# Autodesk Inventor assembly: The_Assembly
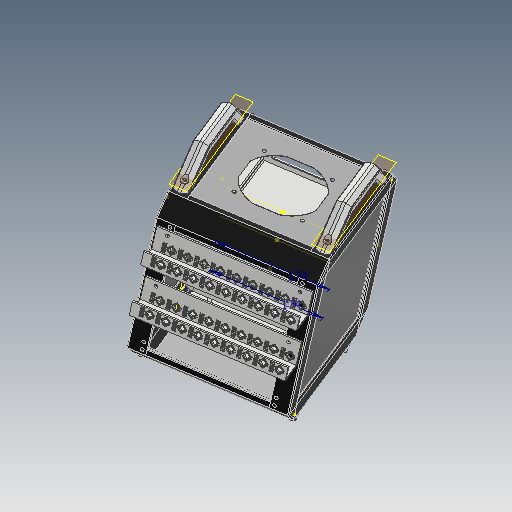
[picture p0: Inventor's stored thumbnail of the model, 512x512]
Saved by Autodesk Inventor 2027 (Build 310192060, 192F)
## iProperties
Created: 2026-07-27
Part Number: The_Assembly
Document SubType Name: Assembly
Designer: prest
Author: prest
## Documents named in this file (17)
- C:\Users\prest\OneDrive\Documents\Projects\Home_Lab_Rack\The_Assembly.iam
- C:\Users\prest\OneDrive\Documents\Projects\Home_Lab_Rack\angles_struts.ipt
- C:\Users\prest\OneDrive\Documents\Projects\Home_Lab_Rack\bottom_edge.ipt
- C:\Users\prest\OneDrive\Documents\Projects\Home_Lab_Rack\horizontal_Edge.ipt
- C:\Users\prest\OneDrive\Documents\Inventor\Content Center Files\R2027\en-US\ANSI B18.3.4M(1)\ANSI B18.3.4M - M6 x 1 x 8(2).ipt
- C:\Users\prest\OneDrive\Documents\Projects\Home_Lab_Rack\mini_PC_mount.ipt
- C:\Users\prest\OneDrive\Documents\Projects\Home_Lab_Rack\router_mount.ipt
- C:\Users\prest\OneDrive\Documents\Projects\Home_Lab_Rack\side_panel_actual.ipt
- C:\Users\prest\OneDrive\Documents\Projects\Home_Lab_Rack\bottom_panel.ipt
- C:\Users\prest\OneDrive\Documents\Projects\Home_Lab_Rack\front_panel_mount_end.ipt
- C:\Users\prest\OneDrive\Documents\Projects\Home_Lab_Rack\top panel.ipt
- C:\Users\prest\OneDrive\Documents\Projects\Home_Lab_Rack\feet.ipt
- C:\Users\prest\OneDrive\Documents\Projects\Home_Lab_Rack\top_edge.ipt
- C:\Users\prest\OneDrive\Documents\Inventor\Content Center Files\R2027\en-US\ASME ANSI B18.3.5M(2)\ASME_ANSI B18.3.5M - M6x20(2).ipt
- C:\Users\prest\OneDrive\Documents\Projects\Home_Lab_Rack\Handle.ipt
- C:\Users\prest\OneDrive\Documents\Inventor\Content Center Files\R2027\en-US\ANSI B18.3.4M(1)\ANSI B18.3.4M - M6 x 1 x 16(2).ipt
- C:\Users\prest\OneDrive\Documents\Projects\Home_Lab_Rack\cable_basket.ipt
## Components (54 placed, 16 different names)
1. Handle:3 — Rigid:21, Rigid:23, Rigid:26
2. Handle:4 — Rigid:22, Rigid:24, Rigid:25
3. Broached Hexagon Socket Button Head Cap Screw - Metric M6 x 1 x 16:1 — Rigid:23
4. Broached Hexagon Socket Button Head Cap Screw - Metric M6 x 1 x 16:2 — Rigid:24
5. Broached Hexagon Socket Button Head Cap Screw - Metric M6 x 1 x 16:3 — Rigid:25
6. Broached Hexagon Socket Button Head Cap Screw - Metric M6 x 1 x 16:4 — Rigid:26
7. cable_basket:1 — Rotational:22, Mate:30
8. cable_basket:2 — Rotational:23, Mate:31
9. Broached Hexagon Socket Flat Countersunk Head Cap Screws - Metric M6x20:1 — Flush:1, Mate:29
10. Broached Hexagon Socket Flat Countersunk Head Cap Screws - Metric M6x20:2 — Mate:27, Mate:28
11. Broached Hexagon Socket Flat Countersunk Head Cap Screws - Metric M6x20:3 — Flush:3, Mate:25
12. Broached Hexagon Socket Flat Countersunk Head Cap Screws - Metric M6x20:4 — Flush:2, Mate:26
13. Broached Hexagon Socket Button Head Cap Screw - Metric M6 x 1 x 8:1 — Rotational:1
14. Broached Hexagon Socket Button Head Cap Screw - Metric M6 x 1 x 8:2 — Rotational:2
15. Broached Hexagon Socket Button Head Cap Screw - Metric M6 x 1 x 8:3 — Rotational:3
16. Broached Hexagon Socket Button Head Cap Screw - Metric M6 x 1 x 8:4 — Rotational:5
17. Broached Hexagon Socket Button Head Cap Screw - Metric M6 x 1 x 8:5 — Rotational:6
18. Broached Hexagon Socket Button Head Cap Screw - Metric M6 x 1 x 8:6 — Rotational:4
19. Broached Hexagon Socket Button Head Cap Screw - Metric M6 x 1 x 8:7 — Rotational:7
20. Broached Hexagon Socket Button Head Cap Screw - Metric M6 x 1 x 8:8 — Rotational:8
21. Broached Hexagon Socket Button Head Cap Screw - Metric M6 x 1 x 8:13 — Rotational:14
22. Broached Hexagon Socket Button Head Cap Screw - Metric M6 x 1 x 8:14 — Rotational:15
23. Broached Hexagon Socket Button Head Cap Screw - Metric M6 x 1 x 8:15 — Rotational:16
24. Broached Hexagon Socket Button Head Cap Screw - Metric M6 x 1 x 8:17 — Rotational:17
25. Broached Hexagon Socket Button Head Cap Screw - Metric M6 x 1 x 8:18 — Rotational:19
26. Broached Hexagon Socket Button Head Cap Screw - Metric M6 x 1 x 8:19 — Rotational:18
27. Broached Hexagon Socket Button Head Cap Screw - Metric M6 x 1 x 8:20 — Rotational:20
28. Broached Hexagon Socket Button Head Cap Screw - Metric M6 x 1 x 8:21 — Rotational:21
29. angles_struts:1 — Rigid:9, Rotational:15, Rotational:16, Rotational:18, Rotational:19, Mate:13, Rigid:16, Mate:19, Mate:20, Mate:22, Mate:24
30. angles_struts:2 — Rigid:10, Rotational:14, Rotational:17, Rotational:20, Rotational:21, Mate:21, Mate:23
31. angles_struts:3 — Rigid:3, Rigid:4, Rigid:5, Rotational:1, Rotational:2, Rotational:5, Rotational:6
32. angles_struts:4 — Rigid:1, Rigid:2, Rigid:6, Rigid:7, Rotational:3, Rotational:4, Rotational:7, Rotational:8, Mate:16
33. horizontal_Edge:1 — Rigid:7, Rigid:9, Mate:1, Mate:2, Mate:4, Mate:5, Mate:8, Mate:11, Mate:14, Mate:17
34. horizontal_Edge:2 — Rigid:4, Rotational:22, Rotational:23
35. horizontal_Edge:3 — Rigid:5, Rigid:10, Mate:30, Mate:31
36. horizontal_Edge:4 — Rigid:6, Mate:3, Mate:6, Mate:7, Mate:9, Mate:10, Mate:12, Mate:15, Mate:18
37. bottom_edge:2 — Rigid:1, Rigid:3, Rigid:17, Rigid:18
38. top panel:1 — Rigid:16
39. bottom_edge:3 — Rigid:2, Rigid:15, Rigid:19, Rigid:20
40. top_edge:1 — Mate:22, Mate:23, Mate:24, Rigid:22, Rigid:28
41. top_edge:2 — Mate:19, Mate:20, Mate:21, Rigid:21, Rigid:27
42. feet:1 — Rigid:18, Mate:27, Mate:28
43. feet:2 — Rigid:17, Flush:1, Mate:29
44. feet:3 — Rigid:20, Flush:2, Mate:26
45. feet:4 — Rigid:19, Flush:3, Mate:25
46. mini_PC_mount:1 — Mate:1, Mate:2, Mate:3
47. mini_PC_mount:2 — Mate:4, Mate:5, Mate:6
48. router_mount:1 — Mate:10, Mate:11, Mate:12
49. router_mount:2 — Mate:7, Mate:8, Mate:9
50. side_panel_actual:2 — Rigid:28
51. bottom_panel:1 — Rigid:15
52. side_panel_actual:1 — Rigid:27
53. front_panel_mount_end:2 — Mate:16, Mate:17, Mate:18
54. front_panel_mount_end:1 — Mate:13, Mate:14, Mate:15
## Relationships (75: Mate 31, WeldJoint 23, RevoluteJoint 18, Flush 3)
- Rigid:1 [WeldJoint]: angles_struts:4 ↔ bottom_edge:2
- Rigid:2 [WeldJoint]: angles_struts:4 ↔ bottom_edge:3
- Rigid:3 [WeldJoint]: angles_struts:3 ↔ bottom_edge:2
- Rigid:4 [WeldJoint]: angles_struts:3 ↔ horizontal_Edge:2
- Rigid:5 [WeldJoint]: angles_struts:3 ↔ horizontal_Edge:3
- Rigid:6 [WeldJoint]: angles_struts:4 ↔ horizontal_Edge:4
- Rigid:7 [WeldJoint]: angles_struts:4 ↔ horizontal_Edge:1
- Rotational:1 [RevoluteJoint]: Broached Hexagon Socket Button Head Cap Screw - Metric M6 x 1 x 8:1 ↔ angles_struts:3
- Rotational:2 [RevoluteJoint]: Broached Hexagon Socket Button Head Cap Screw - Metric M6 x 1 x 8:2 ↔ angles_struts:3
- Rotational:3 [RevoluteJoint]: Broached Hexagon Socket Button Head Cap Screw - Metric M6 x 1 x 8:3 ↔ angles_struts:4
- Rotational:4 [RevoluteJoint]: Broached Hexagon Socket Button Head Cap Screw - Metric M6 x 1 x 8:6 ↔ angles_struts:4
- Rotational:5 [RevoluteJoint]: Broached Hexagon Socket Button Head Cap Screw - Metric M6 x 1 x 8:4 ↔ angles_struts:3
- Rotational:6 [RevoluteJoint]: Broached Hexagon Socket Button Head Cap Screw - Metric M6 x 1 x 8:5 ↔ angles_struts:3
- Rotational:7 [RevoluteJoint]: Broached Hexagon Socket Button Head Cap Screw - Metric M6 x 1 x 8:7 ↔ angles_struts:4
- Rotational:8 [RevoluteJoint]: Broached Hexagon Socket Button Head Cap Screw - Metric M6 x 1 x 8:8 ↔ angles_struts:4
- Rigid:9 [WeldJoint]: angles_struts:1 ↔ horizontal_Edge:1
- Rigid:10 [WeldJoint]: angles_struts:2 ↔ horizontal_Edge:3
- Rotational:14 [RevoluteJoint]: Broached Hexagon Socket Button Head Cap Screw - Metric M6 x 1 x 8:13 ↔ angles_struts:2
- Rotational:15 [RevoluteJoint]: Broached Hexagon Socket Button Head Cap Screw - Metric M6 x 1 x 8:14 ↔ angles_struts:1
- Rotational:16 [RevoluteJoint]: Broached Hexagon Socket Button Head Cap Screw - Metric M6 x 1 x 8:15 ↔ angles_struts:1
- Rotational:17 [RevoluteJoint]: Broached Hexagon Socket Button Head Cap Screw - Metric M6 x 1 x 8:17 ↔ angles_struts:2
- Rotational:18 [RevoluteJoint]: Broached Hexagon Socket Button Head Cap Screw - Metric M6 x 1 x 8:19 ↔ angles_struts:1
- Rotational:19 [RevoluteJoint]: Broached Hexagon Socket Button Head Cap Screw - Metric M6 x 1 x 8:18 ↔ angles_struts:1
- Rotational:20 [RevoluteJoint]: Broached Hexagon Socket Button Head Cap Screw - Metric M6 x 1 x 8:20 ↔ angles_struts:2
- Rotational:21 [RevoluteJoint]: Broached Hexagon Socket Button Head Cap Screw - Metric M6 x 1 x 8:21 ↔ angles_struts:2
- Rigid:15 [WeldJoint]: bottom_edge:3 ↔ bottom_panel:1
- Mate:1: horizontal_Edge:1 ↔ mini_PC_mount:1
- Mate:2: horizontal_Edge:1 ↔ mini_PC_mount:1
- Mate:3: horizontal_Edge:4 ↔ mini_PC_mount:1
- Mate:4: horizontal_Edge:1 ↔ mini_PC_mount:2
- Mate:5: horizontal_Edge:1 ↔ mini_PC_mount:2
- Mate:6: horizontal_Edge:4 ↔ mini_PC_mount:2
- Mate:7: horizontal_Edge:4 ↔ router_mount:2
- Mate:8: horizontal_Edge:1 ↔ router_mount:2
- Mate:9: horizontal_Edge:4 ↔ router_mount:2
- Mate:10: horizontal_Edge:4 ↔ router_mount:1
- Mate:11: horizontal_Edge:1 ↔ router_mount:1
- Mate:12: horizontal_Edge:4 ↔ router_mount:1
- Mate:13: angles_struts:1 ↔ front_panel_mount_end:1
- Mate:14: horizontal_Edge:1 ↔ front_panel_mount_end:1
- Mate:15: horizontal_Edge:4 ↔ front_panel_mount_end:1
- Mate:16: angles_struts:4 ↔ front_panel_mount_end:2
- Mate:17: horizontal_Edge:1 ↔ front_panel_mount_end:2
- Mate:18: horizontal_Edge:4 ↔ front_panel_mount_end:2
- Rigid:16 [WeldJoint]: angles_struts:1 ↔ top panel:1
- Rigid:17 [WeldJoint]: bottom_edge:2 ↔ feet:2
- Rigid:18 [WeldJoint]: bottom_edge:2 ↔ feet:1
- Rigid:19 [WeldJoint]: bottom_edge:3 ↔ feet:4
- Rigid:20 [WeldJoint]: bottom_edge:3 ↔ feet:3
- Mate:19: angles_struts:1 ↔ top_edge:2
- Mate:20: angles_struts:1 ↔ top_edge:2
- Mate:21: angles_struts:2 ↔ top_edge:2
- Mate:22: angles_struts:1 ↔ top_edge:1
- Mate:23: angles_struts:2 ↔ top_edge:1
- Mate:24: angles_struts:1 ↔ top_edge:1
- Flush:1 (-1 mm): Broached Hexagon Socket Flat Countersunk Head Cap Screws - Metric M6x20:1 ↔ feet:2
- Flush:2 (-1 mm): Broached Hexagon Socket Flat Countersunk Head Cap Screws - Metric M6x20:4 ↔ feet:3
- Flush:3 (-1 mm): Broached Hexagon Socket Flat Countersunk Head Cap Screws - Metric M6x20:3 ↔ feet:4
- Mate:25: Broached Hexagon Socket Flat Countersunk Head Cap Screws - Metric M6x20:3 ↔ feet:4
- Mate:26: Broached Hexagon Socket Flat Countersunk Head Cap Screws - Metric M6x20:4 ↔ feet:3
- Mate:27: Broached Hexagon Socket Flat Countersunk Head Cap Screws - Metric M6x20:2 ↔ feet:1
- Mate:28: Broached Hexagon Socket Flat Countersunk Head Cap Screws - Metric M6x20:2 ↔ feet:1
- Mate:29: Broached Hexagon Socket Flat Countersunk Head Cap Screws - Metric M6x20:1 ↔ feet:2
- Rigid:21 [WeldJoint]: Handle:3 ↔ top_edge:2
- Rigid:22 [WeldJoint]: Handle:4 ↔ top_edge:1
- Rigid:23 [WeldJoint]: Handle:3 ↔ Broached Hexagon Socket Button Head Cap Screw - Metric M6 x 1 x 16:1
- Rigid:24 [WeldJoint]: Handle:4 ↔ Broached Hexagon Socket Button Head Cap Screw - Metric M6 x 1 x 16:2
- Rigid:25 [WeldJoint]: Handle:4 ↔ Broached Hexagon Socket Button Head Cap Screw - Metric M6 x 1 x 16:3
- Rigid:26 [WeldJoint]: Handle:3 ↔ Broached Hexagon Socket Button Head Cap Screw - Metric M6 x 1 x 16:4
- Rigid:27 [WeldJoint]: top_edge:2 ↔ side_panel_actual:1
- Rigid:28 [WeldJoint]: top_edge:1 ↔ side_panel_actual:2
- Rotational:22 [RevoluteJoint]: cable_basket:1 ↔ horizontal_Edge:2
- Mate:30: cable_basket:1 ↔ horizontal_Edge:3
- Rotational:23 [RevoluteJoint]: cable_basket:2 ↔ horizontal_Edge:2
- Mate:31: cable_basket:2 ↔ horizontal_Edge:3
